# Autodesk Inventor assembly: assembly_v_2
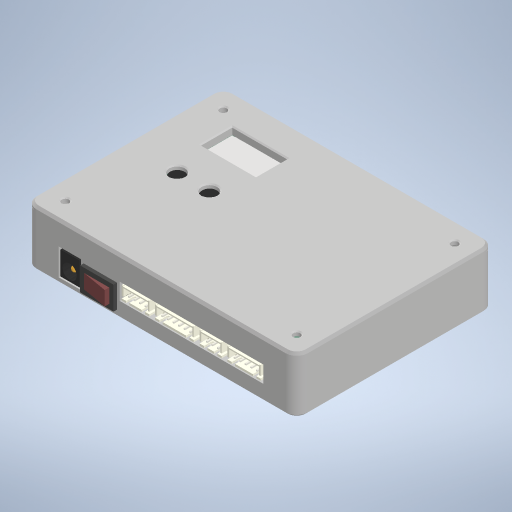
[picture p0: Inventor's stored thumbnail of the model, 512x512]
Saved by Autodesk Inventor 2023 (Build 270158000, 158)
## iProperties
Created: 2023-10-04
Part Number: assembly_v_2
Document SubType Name: Assembly
Designer: mark
Author: mark
## Documents named in this file (5)
- D:\Egyetem\BME MSc\Diplomamunka\opendaq\cad\assembly\v_2\assembly_v_2.iam
- D:\Egyetem\BME MSc\Diplomamunka\opendaq\pcb\opendaq_carrier_1.0\opendaq_carrier_1.0.iam
- D:\Egyetem\BME MSc\Diplomamunka\opendaq\cad\housing\v_2\housing_base_v_2.ipt
- D:\Egyetem\BME MSc\Diplomamunka\opendaq\cad\housing\v_2\housing_top_v_2.ipt
- D:\Egyetem\BME MSc\Diplomamunka\opendaq\cad\misc\rocker_switch.ipt
## Components (4 placed, 4 different names)
1. opendaq_carrier_1.0:1 [sub-assembly] — Mate:1, Mate:2, Mate:3
2. housing_base_v_2:1 — Mate:1, Mate:2, Mate:3, Mate:4, Flush:1, Flush:2, Mate:7, Mate:8, Mate:9
3. housing_top_v_2:1 — Mate:4, Flush:1, Flush:2
4. rocker_switch:1 — Mate:7, Mate:8, Mate:9
## Relationships (9: Mate 7, Flush 2)
- Mate:1: opendaq_carrier_1.0:1 ↔ housing_base_v_2:1
- Mate:2: opendaq_carrier_1.0:1 ↔ housing_base_v_2:1
- Mate:3: opendaq_carrier_1.0:1 ↔ housing_base_v_2:1
- Mate:4: housing_base_v_2:1 ↔ housing_top_v_2:1
- Flush:1: housing_base_v_2:1 ↔ housing_top_v_2:1
- Flush:2: housing_base_v_2:1 ↔ housing_top_v_2:1
- Mate:7: housing_base_v_2:1 ↔ rocker_switch:1
- Mate:8: housing_base_v_2:1 ↔ rocker_switch:1
- Mate:9: housing_base_v_2:1 ↔ rocker_switch:1
